# Autodesk Inventor assembly: estação_bga_3
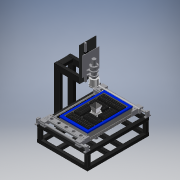
[picture p0: Inventor's stored thumbnail of the model, 180x180]
Saved by Autodesk Inventor 2018 (Build 220112000, 112)
## iProperties
Created: 2018-07-20
Part Number: estação_bga_3
Material: Genérico
Document SubType Name: Assembly
Designer: Usuario
Mass: 28977.3 g
Surface Area: 37496.8 cm^2
Volume: 6730.78 cm^3
Density: 4.30519 g/cm^3
Author: Usuario
## Documents named in this file (12)
- C:\Users\Usuario\Desktop\Estação BGA\Peças 3D\estação_bga_3.iam
- C:\Users\Usuario\Desktop\Estação BGA\Peças 3D\mesa_aquecimento_fresamento.iam
- C:\Users\Usuario\Desktop\Estação BGA\Peças 3D\estrutura.iam
- C:\Users\Usuario\Desktop\Estação BGA\Peças 3D\mesa_suporte_de_placa.iam
- C:\Users\Usuario\Desktop\Estação BGA\Peças 3D\cabeça_inferior.iam
- C:\Users\Usuario\Desktop\Estação BGA\Peças 3D\bocal_inferior.ipt
- C:\Users\Usuario\Desktop\Estação BGA\Peças 3D\ApoioBocalInferior_.ipt
- C:\Users\Usuario\Desktop\Estação BGA\Peças 3D\cabeça_superior_4.iam
- C:\Users\Usuario\Desktop\Estação BGA\Peças 3D\mesa_suporte_de_placa_automatica.iam
- C:\Users\Usuario\Desktop\Estação BGA\Peças 3D\SBR16UU.iam
- C:\Users\Usuario\Desktop\Estação BGA\Peças 3D\Sk16.ipt
- C:\Users\Usuario\Desktop\Estação BGA\Peças 3D\GuiaLinear_16mmx600mm.ipt
## Components (18 placed, 11 different names)
1. mesa_aquecimento_fresamento:1 [sub-assembly] — Coincidência:11, Coincidência:14, Ângulo:1, Coincidência:15, Alinhamento:6, Coincidência:16
2. estrutura:1 [sub-assembly] — Coincidência:6, Alinhamento:2, Coincidência:8, Coincidência:14, Coincidência:17, Alinhamento:7, Alinhamento:8, Coincidência:18, Coincidência:25, Alinhamento:25, Alinhamento:26
3. mesa_suporte_de_placa:1 [sub-assembly] — Coincidência:15, Alinhamento:6, Coincidência:16
4. cabeça_inferior:1 [sub-assembly] — Coincidência:7, Alinhamento:3, Coincidência:9, Coincidência:10, Alinhamento:4, Coincidência:11
5. bocal_inferior:1 — Coincidência:9, Coincidência:10
6. ApoioBocalInferior_:1 — Coincidência:6, Alinhamento:2, Coincidência:7, Alinhamento:3, Coincidência:8, Alinhamento:4, Ângulo:1
7. cabeça_superior_4:1 [sub-assembly] — Coincidência:17, Alinhamento:7, Alinhamento:8
8. mesa_suporte_de_placa_automatica:1 [sub-assembly]
9. SBR16UU:1 [sub-assembly] — Coincidência:28
10. SBR16UU:2 [sub-assembly] — Coincidência:29
11. SBR16UU:3 [sub-assembly] — Coincidência:27
12. SBR16UU:4 [sub-assembly] — Coincidência:26
13. Sk16:1 — Coincidência:22, Alinhamento:17, Alinhamento:22, Alinhamento:26
14. Sk16:2 — Coincidência:21, Alinhamento:18, Alinhamento:22, Alinhamento:23, Coincidência:25, Alinhamento:24, Alinhamento:25
15. Sk16:3 — Coincidência:24, Alinhamento:20, Alinhamento:21, Alinhamento:23, Alinhamento:24
16. Sk16:4 — Alinhamento:19, Coincidência:23, Alinhamento:21
17. GuiaLinear_16mmx600mm:1 — Coincidência:21, Coincidência:22, Alinhamento:17, Alinhamento:18, Coincidência:26, Coincidência:27
18. GuiaLinear_16mmx600mm:2 — Alinhamento:19, Coincidência:23, Coincidência:24, Alinhamento:20, Coincidência:28, Coincidência:29
## Relationships (47: Flush 24, Mate 22, Angle 1)
- Coincidência:6 [Mate]: estrutura:1 ↔ ApoioBocalInferior_:1
- Alinhamento:2 [Flush]: estrutura:1 ↔ ApoioBocalInferior_:1
- Coincidência:7 [Mate]: cabeça_inferior:1 ↔ ApoioBocalInferior_:1
- Alinhamento:3 [Flush] (28 mm): cabeça_inferior:1 ↔ ApoioBocalInferior_:1
- Coincidência:8 [Mate]: estrutura:1 ↔ ApoioBocalInferior_:1
- Coincidência:9 [Mate]: cabeça_inferior:1 ↔ bocal_inferior:1
- Coincidência:10 [Mate]: cabeça_inferior:1 ↔ bocal_inferior:1
- Alinhamento:4 [Flush] (45 mm): cabeça_inferior:1 ↔ ApoioBocalInferior_:1
- Coincidência:11 [Mate]: mesa_aquecimento_fresamento:1 ↔ cabeça_inferior:1
- Coincidência:14 [Mate]: mesa_aquecimento_fresamento:1 ↔ estrutura:1
- Ângulo:1 [Angle] (90 deg): mesa_aquecimento_fresamento:1 ↔ ApoioBocalInferior_:1
- Coincidência:15 [Mate] (17.016 mm): mesa_aquecimento_fresamento:1 ↔ mesa_suporte_de_placa:1
- Alinhamento:6 [Flush]: mesa_aquecimento_fresamento:1 ↔ mesa_suporte_de_placa:1
- Coincidência:16 [Mate] (40.48 mm): mesa_aquecimento_fresamento:1 ↔ mesa_suporte_de_placa:1
- Coincidência:17 [Mate]: estrutura:1 ↔ cabeça_superior_4:1
- Alinhamento:7 [Flush]: estrutura:1 ↔ cabeça_superior_4:1
- Alinhamento:8 [Flush]: estrutura:1 ↔ cabeça_superior_4:1
- Coincidência:18 [Mate]: estrutura:1
- [Flush]: SBR16UU:1 ↔ SBR16UU:2
- [Flush]: SBR16UU:3 ↔ SBR16UU:4
- [Mate]: mesa_suporte_de_placa_automatica:1 ↔ SBR16UU:1
- [Mate]: mesa_suporte_de_placa_automatica:1 ↔ SBR16UU:4
- [Flush]: mesa_suporte_de_placa_automatica:1 ↔ SBR16UU:4
- [Flush]: mesa_suporte_de_placa_automatica:1 ↔ SBR16UU:2
- [Flush]: mesa_suporte_de_placa_automatica:1 ↔ SBR16UU:1
- [Flush]: mesa_suporte_de_placa_automatica:1 ↔ SBR16UU:4
- [Flush]: mesa_suporte_de_placa_automatica:1 ↔ SBR16UU:3
- [Flush]: mesa_suporte_de_placa_automatica:1 ↔ SBR16UU:2
- Coincidência:21 [Mate]: Sk16:2 ↔ GuiaLinear_16mmx600mm:1
- Coincidência:22 [Mate]: Sk16:1 ↔ GuiaLinear_16mmx600mm:1
- Alinhamento:17 [Flush]: Sk16:1 ↔ GuiaLinear_16mmx600mm:1
- Alinhamento:18 [Flush]: Sk16:2 ↔ GuiaLinear_16mmx600mm:1
- Alinhamento:19 [Flush]: Sk16:4 ↔ GuiaLinear_16mmx600mm:2
- Coincidência:23 [Mate]: Sk16:4 ↔ GuiaLinear_16mmx600mm:2
- Coincidência:24 [Mate]: Sk16:3 ↔ GuiaLinear_16mmx600mm:2
- Alinhamento:20 [Flush]: Sk16:3 ↔ GuiaLinear_16mmx600mm:2
- Alinhamento:21 [Flush]: Sk16:3 ↔ Sk16:4
- Alinhamento:22 [Flush]: Sk16:1 ↔ Sk16:2
- Alinhamento:23 [Flush]: Sk16:2 ↔ Sk16:3
- Coincidência:25 [Mate]: estrutura:1 ↔ Sk16:2
- Coincidência:26 [Mate]: SBR16UU:4 ↔ GuiaLinear_16mmx600mm:1
- Coincidência:27 [Mate]: SBR16UU:3 ↔ GuiaLinear_16mmx600mm:1
- Coincidência:28 [Mate]: SBR16UU:1 ↔ GuiaLinear_16mmx600mm:2
- Coincidência:29 [Mate]: SBR16UU:2 ↔ GuiaLinear_16mmx600mm:2
- Alinhamento:24 [Flush]: Sk16:2 ↔ Sk16:3
- Alinhamento:25 [Flush]: estrutura:1 ↔ Sk16:2
- Alinhamento:26 [Flush] (-9.94 mm): estrutura:1 ↔ Sk16:1
## Named parameters: sa_0 = -1.2153e-09, sa_1 = -2.98637e-07, sa_2 = -1000, d56_d18 = 0 mm, d57_d19 = 0 mm, d62_d26 = 0 mm, d63_d27 = 0 mm, d64_d28 = 0 mm, d65_d29 = 0 mm
note: some values were not read from the file. Shown as the stored number, unit unknown: "sa_0", "sa_1", "sa_2".
